# Autodesk Inventor assembly: Top_Backboard Assy
(part 2 of 2)
- [Mate] (8 mm): Socket Cap Screw - Standard - (A2) - M4 x 16:17 ↔ Nyloc Nut - M4:35
- [Mate] (18 mm): Socket Cap Screw - Standard - (A2) - M4 x 25:18 ↔ Nyloc Nut - M4:34
- [Mate]: Socket Cap Screw - Standard - (A2) - M4 x 25:18 ↔ Top_Angle Bracket:9
- [Mate]: Socket Cap Screw - Standard - (A2) - M4 x 25:18 ↔ Top_Angle Bracket:9
- [Mate]: Top_Angle Bracket:9 ↔ Socket Cap Screw - Standard - (A2) - M4 x 25:17
- [Mate]: Top_Angle Bracket:9 ↔ Socket Cap Screw - Standard - (A2) - M4 x 25:17
- [Mate]: Socket Cap Screw - Standard - (A2) - M4 x 16:17 ↔ Top_Angle Bracket:9
- [Mate]: Top_Angle Bracket:9 ↔ Socket Cap Screw - Standard - (A2) - M4 x 16:18
- [Mate]: Socket Cap Screw - Standard - (A2) - M4 x 16:17 ↔ Top_Angle Bracket:9
- [Mate]: Top_Angle Bracket:9 ↔ Socket Cap Screw - Standard - (A2) - M4 x 16:18
- [Mate]: Socket Cap Screw - Standard - (A2) - M4 x 25:19 ↔ Nyloc Nut - M4:37
- [Mate]: Socket Cap Screw - Standard - (A2) - M4 x 25:20 ↔ Nyloc Nut - M4:38
- [Mate]: Nyloc Nut - M4:39 ↔ Socket Cap Screw - Standard - (A2) - M4 x 16:19
- [Mate]: Nyloc Nut - M4:40 ↔ Socket Cap Screw - Standard - (A2) - M4 x 16:20
- [Mate] (18 mm): Socket Cap Screw - Standard - (A2) - M4 x 25:19 ↔ Nyloc Nut - M4:37
- [Mate] (8 mm): Nyloc Nut - M4:40 ↔ Socket Cap Screw - Standard - (A2) - M4 x 16:20
- [Mate] (8 mm): Nyloc Nut - M4:39 ↔ Socket Cap Screw - Standard - (A2) - M4 x 16:19
- [Mate] (18 mm): Socket Cap Screw - Standard - (A2) - M4 x 25:20 ↔ Nyloc Nut - M4:38
- [Mate]: Top_Angle Bracket:10 ↔ Socket Cap Screw - Standard - (A2) - M4 x 25:20
- [Mate]: Top_Angle Bracket:10 ↔ Socket Cap Screw - Standard - (A2) - M4 x 25:20
- [Mate]: Top_Angle Bracket:10 ↔ Socket Cap Screw - Standard - (A2) - M4 x 25:19
- [Mate]: Top_Angle Bracket:10 ↔ Socket Cap Screw - Standard - (A2) - M4 x 25:19
- [Mate]: Top_Angle Bracket:10 ↔ Socket Cap Screw - Standard - (A2) - M4 x 16:19
- [Mate]: Socket Cap Screw - Standard - (A2) - M4 x 16:20 ↔ Top_Angle Bracket:10
- [Mate]: Top_Angle Bracket:10 ↔ Socket Cap Screw - Standard - (A2) - M4 x 16:19
- [Mate]: Socket Cap Screw - Standard - (A2) - M4 x 16:20 ↔ Top_Angle Bracket:10
- [Mate]: Socket Cap Screw - Standard - (A2) - M4 x 25:21 ↔ Nyloc Nut - M4:41
- [Mate]: Socket Cap Screw - Standard - (A2) - M4 x 25:22 ↔ Nyloc Nut - M4:42
- [Mate]: Socket Cap Screw - Standard - (A2) - M4 x 16:21 ↔ Nyloc Nut - M4:43
- [Mate]: Socket Cap Screw - Standard - (A2) - M4 x 16:22 ↔ Nyloc Nut - M4:44
- [Mate] (18 mm): Socket Cap Screw - Standard - (A2) - M4 x 25:21 ↔ Nyloc Nut - M4:41
- [Mate] (8 mm): Socket Cap Screw - Standard - (A2) - M4 x 16:22 ↔ Nyloc Nut - M4:44
- [Mate] (8 mm): Socket Cap Screw - Standard - (A2) - M4 x 16:21 ↔ Nyloc Nut - M4:43
- [Mate] (18 mm): Socket Cap Screw - Standard - (A2) - M4 x 25:22 ↔ Nyloc Nut - M4:42
- [Mate]: Socket Cap Screw - Standard - (A2) - M4 x 25:22 ↔ Top_Angle Bracket:11
- [Mate]: Socket Cap Screw - Standard - (A2) - M4 x 25:22 ↔ Top_Angle Bracket:11
- [Mate]: Top_Angle Bracket:11 ↔ Socket Cap Screw - Standard - (A2) - M4 x 25:21
- [Mate]: Top_Angle Bracket:11 ↔ Socket Cap Screw - Standard - (A2) - M4 x 25:21
- [Mate]: Socket Cap Screw - Standard - (A2) - M4 x 16:21 ↔ Top_Angle Bracket:11
- [Mate]: Top_Angle Bracket:11 ↔ Socket Cap Screw - Standard - (A2) - M4 x 16:22
- [Mate]: Socket Cap Screw - Standard - (A2) - M4 x 16:21 ↔ Top_Angle Bracket:11
- [Mate]: Top_Angle Bracket:11 ↔ Socket Cap Screw - Standard - (A2) - M4 x 16:22
- [Mate]: Nyloc Nut - M4:45 ↔ Socket Cap Screw - Standard - (A2) - M4 x 25:23
- [Mate]: Nyloc Nut - M4:46 ↔ Socket Cap Screw - Standard - (A2) - M4 x 25:24
- [Mate]: Nyloc Nut - M4:47 ↔ Socket Cap Screw - Standard - (A2) - M4 x 16:23
- [Mate]: Nyloc Nut - M4:48 ↔ Socket Cap Screw - Standard - (A2) - M4 x 16:24
- [Mate] (18 mm): Nyloc Nut - M4:45 ↔ Socket Cap Screw - Standard - (A2) - M4 x 25:23
- [Mate] (8 mm): Nyloc Nut - M4:48 ↔ Socket Cap Screw - Standard - (A2) - M4 x 16:24
- [Mate] (8 mm): Nyloc Nut - M4:47 ↔ Socket Cap Screw - Standard - (A2) - M4 x 16:23
- [Mate] (18 mm): Nyloc Nut - M4:46 ↔ Socket Cap Screw - Standard - (A2) - M4 x 25:24
- [Mate]: Top_Angle Bracket:12 ↔ Socket Cap Screw - Standard - (A2) - M4 x 25:24
- [Mate]: Top_Angle Bracket:12 ↔ Socket Cap Screw - Standard - (A2) - M4 x 25:24
- [Mate]: Top_Angle Bracket:12 ↔ Socket Cap Screw - Standard - (A2) - M4 x 25:23
- [Mate]: Top_Angle Bracket:12 ↔ Socket Cap Screw - Standard - (A2) - M4 x 25:23
- [Mate]: Top_Angle Bracket:12 ↔ Socket Cap Screw - Standard - (A2) - M4 x 16:23
- [Mate]: Top_Angle Bracket:12 ↔ Socket Cap Screw - Standard - (A2) - M4 x 16:24
- [Mate]: Top_Angle Bracket:12 ↔ Socket Cap Screw - Standard - (A2) - M4 x 16:23
- [Mate]: Top_Angle Bracket:12 ↔ Socket Cap Screw - Standard - (A2) - M4 x 16:24
- [Mate]: Socket Cap Screw - Standard - (A2) - M4 x 25:25 ↔ Nyloc Nut - M4:49
- [Mate]: Socket Cap Screw - Standard - (A2) - M4 x 25:26 ↔ Nyloc Nut - M4:50
- [Mate]: Nyloc Nut - M4:51 ↔ Socket Cap Screw - Standard - (A2) - M4 x 16:25
- [Mate]: Nyloc Nut - M4:52 ↔ Socket Cap Screw - Standard - (A2) - M4 x 16:26
- [Mate] (18 mm): Socket Cap Screw - Standard - (A2) - M4 x 25:25 ↔ Nyloc Nut - M4:49
- [Mate] (8 mm): Nyloc Nut - M4:52 ↔ Socket Cap Screw - Standard - (A2) - M4 x 16:26
- [Mate] (8 mm): Nyloc Nut - M4:51 ↔ Socket Cap Screw - Standard - (A2) - M4 x 16:25
- [Mate] (18 mm): Socket Cap Screw - Standard - (A2) - M4 x 25:26 ↔ Nyloc Nut - M4:50
- [Mate]: Top_Angle Bracket:13 ↔ Socket Cap Screw - Standard - (A2) - M4 x 25:26
- [Mate]: Top_Angle Bracket:13 ↔ Socket Cap Screw - Standard - (A2) - M4 x 25:26
- [Mate]: Socket Cap Screw - Standard - (A2) - M4 x 25:25 ↔ Top_Angle Bracket:13
- [Mate]: Socket Cap Screw - Standard - (A2) - M4 x 25:25 ↔ Top_Angle Bracket:13
- [Mate]: Top_Angle Bracket:13 ↔ Socket Cap Screw - Standard - (A2) - M4 x 16:25
- [Mate]: Socket Cap Screw - Standard - (A2) - M4 x 16:26 ↔ Top_Angle Bracket:13
- [Mate]: Top_Angle Bracket:13 ↔ Socket Cap Screw - Standard - (A2) - M4 x 16:25
- [Mate]: Socket Cap Screw - Standard - (A2) - M4 x 16:26 ↔ Top_Angle Bracket:13
- [Mate]: Socket Cap Screw - Standard - (A2) - M4 x 25:27 ↔ Nyloc Nut - M4:53
- [Mate]: Socket Cap Screw - Standard - (A2) - M4 x 25:28 ↔ Nyloc Nut - M4:54
- [Mate]: Socket Cap Screw - Standard - (A2) - M4 x 16:27 ↔ Nyloc Nut - M4:55
- [Mate]: Socket Cap Screw - Standard - (A2) - M4 x 16:28 ↔ Nyloc Nut - M4:56
- [Mate] (18 mm): Socket Cap Screw - Standard - (A2) - M4 x 25:27 ↔ Nyloc Nut - M4:53
- [Mate] (8 mm): Socket Cap Screw - Standard - (A2) - M4 x 16:28 ↔ Nyloc Nut - M4:56
- [Mate] (8 mm): Socket Cap Screw - Standard - (A2) - M4 x 16:27 ↔ Nyloc Nut - M4:55
- [Mate] (18 mm): Socket Cap Screw - Standard - (A2) - M4 x 25:28 ↔ Nyloc Nut - M4:54
- [Mate]: Top_Angle Bracket:14 ↔ Socket Cap Screw - Standard - (A2) - M4 x 25:28
- [Mate]: Top_Angle Bracket:14 ↔ Socket Cap Screw - Standard - (A2) - M4 x 25:28
- [Mate]: Top_Angle Bracket:14 ↔ Socket Cap Screw - Standard - (A2) - M4 x 25:27
- [Mate]: Top_Angle Bracket:14 ↔ Socket Cap Screw - Standard - (A2) - M4 x 25:27
- [Mate]: Top_Angle Bracket:14 ↔ Socket Cap Screw - Standard - (A2) - M4 x 16:27
- [Mate]: Top_Angle Bracket:14 ↔ Socket Cap Screw - Standard - (A2) - M4 x 16:28
- [Mate]: Top_Angle Bracket:14 ↔ Socket Cap Screw - Standard - (A2) - M4 x 16:27
- [Mate]: Top_Angle Bracket:14 ↔ Socket Cap Screw - Standard - (A2) - M4 x 16:28
- Mate:320: Top_Backboard:1 ↔ Top_Angle Bracket:1
- Mate:321: Top_Backboard:1 ↔ Socket Cap Screw - Standard - (A2) - M4 x 25:1
- Mate:322: Top_Backboard:1 ↔ Socket Cap Screw - Standard - (A2) - M4 x 25:2
- Mate:323: Top_Backboard:1 ↔ Top_Angle Bracket:2
- Mate:324: Top_Backboard:1 ↔ Top_Angle Bracket:3
- Mate:325: Top_Backboard:1 ↔ Top_Angle Bracket:4
- Mate:326: Top_Backboard:1 ↔ Top_Angle Bracket:5
- Mate:327: Top_Backboard:1 ↔ Top_Angle Bracket:6
- Mate:328: Top_Backboard:1 ↔ Top_Angle Bracket:7
- Mate:329: Top_Backboard:1 ↔ Top_Angle Bracket:8
- Mate:330: Top_Backboard:1 ↔ Top_Angle Bracket:9
- Mate:331: Top_Backboard:1 ↔ Top_Angle Bracket:10
- Mate:332: Top_Backboard:1 ↔ Top_Angle Bracket:11
- Mate:333: Top_Backboard:1 ↔ Top_Angle Bracket:12
- Mate:334: Top_Backboard:1 ↔ Top_Angle Bracket:13
- Mate:335: Top_Backboard:1 ↔ Top_Angle Bracket:14
- Mate:336: Top_Backboard:1 ↔ Socket Cap Screw - Standard - (A2) - M4 x 25:3
- Mate:337: Top_Backboard:1 ↔ Socket Cap Screw - Standard - (A2) - M4 x 25:4
- Mate:338: Top_Backboard:1 ↔ Socket Cap Screw - Standard - (A2) - M4 x 25:5
- Mate:339: Top_Backboard:1 ↔ Socket Cap Screw - Standard - (A2) - M4 x 25:6
- Mate:340: Top_Backboard:1 ↔ Socket Cap Screw - Standard - (A2) - M4 x 25:7
- Mate:341: Top_Backboard:1 ↔ Socket Cap Screw - Standard - (A2) - M4 x 25:8
- Mate:342: Top_Backboard:1 ↔ Socket Cap Screw - Standard - (A2) - M4 x 25:9
- Mate:343: Top_Backboard:1 ↔ Socket Cap Screw - Standard - (A2) - M4 x 25:10
- Mate:344: Top_Backboard:1 ↔ Socket Cap Screw - Standard - (A2) - M4 x 25:11
- Mate:345: Top_Backboard:1 ↔ Socket Cap Screw - Standard - (A2) - M4 x 25:12
- Mate:346: Top_Backboard:1 ↔ Socket Cap Screw - Standard - (A2) - M4 x 25:23
- Mate:347: Top_Backboard:1 ↔ Socket Cap Screw - Standard - (A2) - M4 x 25:24
- Mate:348: Top_Backboard:1 ↔ Socket Cap Screw - Standard - (A2) - M4 x 25:13
- Mate:349: Top_Backboard:1 ↔ Socket Cap Screw - Standard - (A2) - M4 x 25:14
- Mate:350: Top_Backboard:1 ↔ Socket Cap Screw - Standard - (A2) - M4 x 25:15
- Mate:351: Top_Backboard:1 ↔ Socket Cap Screw - Standard - (A2) - M4 x 25:16
- Mate:352: Top_Backboard:1 ↔ Socket Cap Screw - Standard - (A2) - M4 x 25:17
- Mate:353: Top_Backboard:1 ↔ Socket Cap Screw - Standard - (A2) - M4 x 25:18
- Mate:354: Top_Backboard:1 ↔ Socket Cap Screw - Standard - (A2) - M4 x 25:19
- Mate:355: Top_Backboard:1 ↔ Socket Cap Screw - Standard - (A2) - M4 x 25:20
- Mate:356: Top_Backboard:1 ↔ Socket Cap Screw - Standard - (A2) - M4 x 25:21
- Mate:357: Top_Backboard:1 ↔ Socket Cap Screw - Standard - (A2) - M4 x 25:22
- Mate:358: Top_Backboard:1 ↔ Socket Cap Screw - Standard - (A2) - M4 x 25:25
- Mate:359: Top_Backboard:1 ↔ Socket Cap Screw - Standard - (A2) - M4 x 25:26
- Mate:360: Top_Backboard:1 ↔ Socket Cap Screw - Standard - (A2) - M4 x 25:27
- Mate:361: Top_Backboard:1 ↔ Socket Cap Screw - Standard - (A2) - M4 x 25:28
- Mate:362: Top_Backboard:1 ↔ Top_Reinforcement_LHS:1
- Mate:363: Top_Backboard:1 ↔ Top_Reinforcement_RHS:1
- Mate:364: Top_Backboard:1 ↔ Top_Reinforcement 2:2
- Mate:365: Top_Backboard:1 ↔ Top_Reinforcement 2:3
- Mate:366: Top_Backboard:1 ↔ Top_Reinforcement 2:1
- Mate:367: Top_Backboard:1 ↔ Din97 - 4x25 - Steel Wood Screw:1
- Flush:29: Top_Backboard:1 ↔ Din97 - 4x25 - Steel Wood Screw:1
- Mate:368: Top_Backboard:1 ↔ Din97 - 4x25 - Steel Wood Screw:2
- Flush:30: Top_Backboard:1 ↔ Din97 - 4x25 - Steel Wood Screw:2
- Mate:369: Top_Backboard:1 ↔ Din97 - 4x25 - Steel Wood Screw:3
- Mate:370: Top_Backboard:1 ↔ Din97 - 4x25 - Steel Wood Screw:5
- Mate:371: Top_Backboard:1 ↔ Din97 - 4x25 - Steel Wood Screw:4
- Flush:31: Top_Backboard:1 ↔ Din97 - 4x25 - Steel Wood Screw:3
- Flush:32: Top_Backboard:1 ↔ Din97 - 4x25 - Steel Wood Screw:4
- Flush:33: Top_Backboard:1 ↔ Din97 - 4x25 - Steel Wood Screw:5
- [Mate]: Nyloc Nut - M4:81 ↔ Socket Cap Screw - Standard - (A2) - M4 x 20:1
- [Mate]: Nyloc Nut - M4:82 ↔ Socket Cap Screw - Standard - (A2) - M4 x 20:4
- Mate:374 (13 mm): Nyloc Nut - M4:82 ↔ Socket Cap Screw - Standard - (A2) - M4 x 20:4
- Mate:375 (13 mm): Nyloc Nut - M4:81 ↔ Socket Cap Screw - Standard - (A2) - M4 x 20:1
- [Mate]: Top_Angle Bracket:21 ↔ Socket Cap Screw - Standard - (A2) - M4 x 20:1
- [Mate]: Top_Angle Bracket:21 ↔ Socket Cap Screw - Standard - (A2) - M4 x 20:4
- [Mate]: Top_Angle Bracket:21 ↔ Socket Cap Screw - Standard - (A2) - M4 x 20:1
- [Mate]: Top_Angle Bracket:21 ↔ Socket Cap Screw - Standard - (A2) - M4 x 20:4
- [Mate]: Nyloc Nut - M4:83 ↔ Socket Cap Screw - Standard - (A2) - M4 x 20:7
- [Mate]: Nyloc Nut - M4:84 ↔ Socket Cap Screw - Standard - (A2) - M4 x 20:10
- Mate:386 (13 mm): Nyloc Nut - M4:84 ↔ Socket Cap Screw - Standard - (A2) - M4 x 20:10
- Mate:387 (13 mm): Nyloc Nut - M4:83 ↔ Socket Cap Screw - Standard - (A2) - M4 x 20:7
- [Mate]: Top_Angle Bracket:22 ↔ Socket Cap Screw - Standard - (A2) - M4 x 20:7
- [Mate]: Top_Angle Bracket:22 ↔ Socket Cap Screw - Standard - (A2) - M4 x 20:10
- [Mate]: Top_Angle Bracket:22 ↔ Socket Cap Screw - Standard - (A2) - M4 x 20:7
- [Mate]: Top_Angle Bracket:22 ↔ Socket Cap Screw - Standard - (A2) - M4 x 20:10
- Mate:396: Top_Backboard:1 ↔ Top_Angle Bracket:21
- Mate:397: Top_Backboard:1 ↔ Top_Angle Bracket:21
- Mate:398: Top_Backboard:1 ↔ Top_Angle Bracket:21
- Mate:399: Top_Backboard:1 ↔ Top_Angle Bracket:22
- Mate:400: Top_Backboard:1 ↔ Top_Angle Bracket:22
- Mate:401: Top_Backboard:1 ↔ Top_Angle Bracket:22
- Flush:34: Socket Cap Screw - Standard - (A2) - M4 x 16:45 ↔ Socket Cap Screw - Standard - (A2) - M4 x 16:46
- Mate:402: Top_Angle Bracket:21 ↔ Socket Cap Screw - Standard - (A2) - M4 x 16:45
- Mate:403: Top_Angle Bracket:21 ↔ Socket Cap Screw - Standard - (A2) - M4 x 16:45
- Mate:404: Top_Angle Bracket:21 ↔ Socket Cap Screw - Standard - (A2) - M4 x 16:46
- [Flush]: Socket Cap Screw - Standard - (A2) - M4 x 16:47 ↔ Socket Cap Screw - Standard - (A2) - M4 x 16:48
- Mate:405: Top_Angle Bracket:22 ↔ Socket Cap Screw - Standard - (A2) - M4 x 16:47
- Mate:406: Top_Angle Bracket:22 ↔ Socket Cap Screw - Standard - (A2) - M4 x 16:48
- Mate:407: Top_Angle Bracket:22 ↔ Socket Cap Screw - Standard - (A2) - M4 x 16:47
## Named parameters: d66_d33 = 0 mm, d67_d34 = 0 mm, d68_d35 = 0 mm, d69_d36 = 0 mm, d70_d33 = 0 mm, d71_d34 = 0 mm, d72_d35 = 0 mm, d73_d36 = 0 mm, d74_d33 = 0 mm, d75_d34 = 0 mm, d76_d35 = 0 mm, d77_d36 = 0 mm, d143_d133 = 8 mm, d144_d134 = 18 mm, d145_d135 = 0 mm, d146_d136 = 0 mm, d147_d137 = 0 mm, d148_d138 = 0 mm, d149_d139 = 0 mm, d150_d140 = 0 mm, d151_d141 = 0 mm, d152_d142 = 0 mm, d153_d69 = 0 mm, d154_d70 = 0 mm, d155_d71 = 0 mm, d156_d72 = 0 mm, d157_d131 = 18 mm, d158_d132 = 8 mm, d159_d133 = 8 mm, d160_d134 = 18 mm, d161_d135 = 0 mm, d162_d136 = 0 mm, d163_d137 = 0 mm, d164_d138 = 0 mm, d165_d139 = 0 mm, d166_d140 = 0 mm, d167_d141 = 0 mm, d168_d142 = 0 mm, d169_d69 = 0 mm, d170_d70 = 0 mm, d171_d71 = 0 mm, d172_d72 = 0 mm, d173_d131 = 18 mm, d174_d132 = 8 mm, d175_d133 = 8 mm, d176_d134 = 18 mm, d177_d135 = 0 mm, d178_d136 = 0 mm, d179_d137 = 0 mm, d180_d138 = 0 mm, d181_d139 = 0 mm, d182_d140 = 0 mm, d183_d141 = 0 mm, d184_d142 = 0 mm, d185_d69 = 0 mm, d186_d70 = 0 mm, d187_d71 = 0 mm, d188_d72 = 0 mm, d189_d131 = 18 mm, d190_d132 = 8 mm, d191_d133 = 8 mm, d192_d134 = 18 mm, d193_d135 = 0 mm, d194_d136 = 0 mm, d195_d137 = 0 mm, d196_d138 = 0 mm, d197_d139 = 0 mm, d198_d140 = 0 mm, d199_d141 = 0 mm, d200_d142 = 0 mm, d201_d69 = 0 mm, d202_d70 = 0 mm, d203_d71 = 0 mm, d204_d72 = 0 mm, d205_d131 = 18 mm, d206_d132 = 8 mm, d207_d133 = 8 mm, d208_d134 = 18 mm, d209_d135 = 0 mm, d210_d136 = 0 mm, d211_d137 = 0 mm, d212_d138 = 0 mm, d213_d139 = 0 mm, d214_d140 = 0 mm, d215_d141 = 0 mm, d216_d142 = 0 mm, d217_d69 = 0 mm, d218_d70 = 0 mm, d219_d71 = 0 mm, d220_d72 = 0 mm, d221_d131 = 18 mm, d222_d132 = 8 mm, d223_d133 = 8 mm, d224_d134 = 18 mm, d225_d135 = 0 mm, d226_d136 = 0 mm, d227_d137 = 0 mm, d228_d138 = 0 mm, d229_d139 = 0 mm, d230_d140 = 0 mm, d231_d141 = 0 mm, d232_d142 = 0 mm, d233_d69 = 0 mm, d234_d70 = 0 mm, d235_d71 = 0 mm, d236_d72 = 0 mm, d237_d131 = 18 mm, d238_d132 = 8 mm, d239_d133 = 8 mm, d240_d134 = 18 mm, d241_d135 = 0 mm, d242_d136 = 0 mm, d243_d137 = 0 mm, d244_d138 = 0 mm, d245_d139 = 0 mm, d246_d140 = 0 mm, d247_d141 = 0 mm, d248_d142 = 0 mm, d249_d69 = 0 mm, d250_d70 = 0 mm, d251_d71 = 0 mm, d252_d72 = 0 mm, d253_d131 = 18 mm, d254_d132 = 8 mm, d255_d133 = 8 mm, d256_d134 = 18 mm, d257_d135 = 0 mm, d258_d136 = 0 mm, d259_d137 = 0 mm, d260_d138 = 0 mm, d261_d139 = 0 mm, d262_d140 = 0 mm, d263_d141 = 0 mm, d264_d142 = 0 mm, d265_d69 = 0 mm, d266_d70 = 0 mm, d267_d71 = 0 mm, d268_d72 = 0 mm, d269_d131 = 18 mm, d270_d132 = 8 mm, d271_d133 = 8 mm, d272_d134 = 18 mm, d273_d135 = 0 mm, d274_d136 = 0 mm, d275_d137 = 0 mm, d276_d138 = 0 mm, d277_d139 = 0 mm, d278_d140 = 0 mm, d279_d141 = 0 mm, d280_d142 = 0 mm, d281_d69 = 0 mm, d282_d70 = 0 mm, d283_d71 = 0 mm, d284_d72 = 0 mm, d285_d131 = 18 mm, d286_d132 = 8 mm, d287_d133 = 8 mm, d288_d134 = 18 mm, d289_d135 = 0 mm, d290_d136 = 0 mm, d291_d137 = 0 mm, d292_d138 = 0 mm, d293_d139 = 0 mm, d294_d140 = 0 mm, d295_d141 = 0 mm, d296_d142 = 0 mm, d297_d69 = 0 mm, d298_d70 = 0 mm, d299_d71 = 0 mm, d300_d72 = 0 mm, d301_d131 = 18 mm, d302_d132 = 8 mm, d303_d133 = 8 mm, d304_d134 = 18 mm, d305_d135 = 0 mm, d306_d136 = 0 mm, d307_d137 = 0 mm, d308_d138 = 0 mm, d309_d139 = 0 mm, d310_d140 = 0 mm, d311_d141 = 0 mm, d312_d142 = 0 mm, d313_d69 = 0 mm, d314_d70 = 0 mm, d315_d71 = 0 mm, d316_d72 = 0 mm, d317_d131 = 18 mm, d318_d132 = 8 mm, d319_d133 = 8 mm, d320_d134 = 18 mm, d321_d135 = 0 mm, d322_d136 = 0 mm, d323_d137 = 0 mm, d324_d138 = 0 mm, d325_d139 = 0 mm, d326_d140 = 0 mm, d327_d141 = 0 mm, d328_d142 = 0 mm, d329_d69 = 0 mm, d330_d70 = 0 mm, d331_d71 = 0 mm, d332_d72 = 0 mm, d333_d131 = 18 mm, d334_d132 = 8 mm, d335_d133 = 8 mm, d336_d134 = 18 mm, d337_d135 = 0 mm, d338_d136 = 0 mm, d339_d137 = 0 mm, d340_d138 = 0 mm, d341_d139 = 0 mm, d342_d140 = 0 mm, d343_d141 = 0 mm, d344_d142 = 0 mm, d345_d69 = 0 mm, d346_d70 = 0 mm, d347_d71 = 0 mm, d348_d72 = 0 mm, d349_d131 = 18 mm, d350_d132 = 8 mm, d452_d143_d133 = 13 mm, d457_d149_d139 = 0 mm, d458_d150_d140 = 0 mm, d459_d151_d141 = 0 mm, d460_d152_d142 = 0 mm, d461_d155_d71 = 0 mm, d462_d156_d72 = 0 mm, d463_d158_d132 = 13 mm, d464_d143_d133 = 13 mm, d469_d149_d139 = 0 mm, d470_d150_d140 = 0 mm, d471_d151_d141 = 0 mm, d472_d152_d142 = 0 mm, d473_d155_d71 = 0 mm, d474_d156_d72 = 0 mm, d475_d158_d132 = 13 mm, d486_d482 = 0 mm
